# Autodesk Inventor assembly: Truss
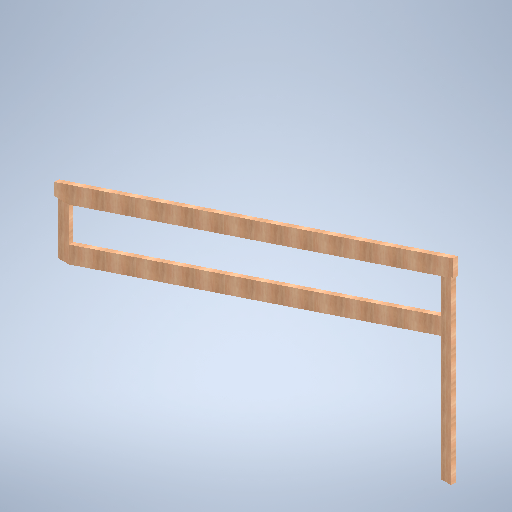
[picture p0: Inventor's stored thumbnail of the model, 512x512]
Saved by Autodesk Inventor 2025 (Build 290162010, 162A)
## iProperties
Created: 2024-09-16
Part Number: Truss
Document SubType Name: Assembly
Designer: Tom
Author: Tom
## Documents named in this file (6)
- C:\Users\Tom\Documents\Inventor\Mobility\Additional_Building\Truss.iam
- C:\Users\Tom\Documents\Inventor\Mobility\Additional_Building\Rafter.ipt
- C:\Users\Tom\Documents\Inventor\Mobility\Additional_Building\Stud_With_Height_60.28125_Inches.ipt
- C:\Users\Tom\Documents\Inventor\Mobility\Additional_Building\Mending_Plate.ipt
- C:\Users\Tom\Documents\Inventor\Mobility\Additional_Building\Stud_With_Height_17.40625_Inches.ipt
- C:\Users\Tom\Documents\Inventor\Mobility\Additional_Building\Ceiling_Joist.ipt
## Components (12 placed, 5 different names)
1. Rafter:1 — Mate:1, Flush:1, Flush:2, Mate:4, Flush:4, Flush:5, Flush:6, Mate:6, Flush:9, Mate:7
2. Stud_With_Height_60.28125_Inches:1 — Mate:4, Flush:4, Flush:5, Flush:10, Flush:11, Mate:9, Flush:14, Flush:15
3. Stud_With_Height_17.40625_Inches:1 — Mate:1, Flush:1, Flush:2, Mate:2, Mate:3, Flush:3, Mate:5, Flush:8, Flush:12, Flush:13
4. Ceiling_Joist:1 — Flush:6, Mate:5, Flush:7, Mate:8
5. Mending_Plate:1 — Mate:6, Flush:8, Flush:9
6. Mending_Plate:3 — Mate:8, Flush:12, Flush:13
7. Mending_Plate:2 — Mate:7, Flush:10, Flush:11
8. Mending_Plate:4 — Mate:9, Flush:14, Flush:15
9. Mending_Plate:5
10. Mending_Plate:6
11. Mending_Plate:7
12. Mending_Plate:8
## Component patterns: (2 elements, first: Mending_Plate:1 + Mending_Plate:3 + Mending_Plate:2 + Mending_Plate:4)
## Relationships (24: Flush 15, Mate 9)
- Mate:1: Rafter:1 ↔ Stud_With_Height_17.40625_Inches:1
- Flush:1: Rafter:1 ↔ Stud_With_Height_17.40625_Inches:1
- Flush:2 (34.925 mm): Rafter:1 ↔ Stud_With_Height_17.40625_Inches:1
- Mate:2: Stud_With_Height_17.40625_Inches:1
- Mate:3: Stud_With_Height_17.40625_Inches:1
- Flush:3: Stud_With_Height_17.40625_Inches:1
- Mate:4: Rafter:1 ↔ Stud_With_Height_60.28125_Inches:1
- Flush:4: Rafter:1 ↔ Stud_With_Height_60.28125_Inches:1
- Flush:5: Rafter:1 ↔ Stud_With_Height_60.28125_Inches:1
- Flush:6: Rafter:1 ↔ Ceiling_Joist:1
- Mate:5: Stud_With_Height_17.40625_Inches:1 ↔ Ceiling_Joist:1
- Flush:7: Ceiling_Joist:1
- Mate:6: Rafter:1 ↔ Mending_Plate:1
- Flush:8 (6.35 mm): Stud_With_Height_17.40625_Inches:1 ↔ Mending_Plate:1
- Flush:9 (-76.2 mm): Rafter:1 ↔ Mending_Plate:1
- Mate:7: Rafter:1 ↔ Mending_Plate:2
- Flush:10 (6.35 mm): Stud_With_Height_60.28125_Inches:1 ↔ Mending_Plate:2
- Flush:11 (1401.7625 mm): Stud_With_Height_60.28125_Inches:1 ↔ Mending_Plate:2
- Mate:8: Ceiling_Joist:1 ↔ Mending_Plate:3
- Flush:12: Stud_With_Height_17.40625_Inches:1 ↔ Mending_Plate:3
- Flush:13 (44.45 mm): Stud_With_Height_17.40625_Inches:1 ↔ Mending_Plate:3
- Mate:9: Stud_With_Height_60.28125_Inches:1 ↔ Mending_Plate:4
- Flush:14 (1057.275 mm): Stud_With_Height_60.28125_Inches:1 ↔ Mending_Plate:4
- Flush:15: Stud_With_Height_60.28125_Inches:1 ↔ Mending_Plate:4
